# Autodesk Inventor assembly: Claw
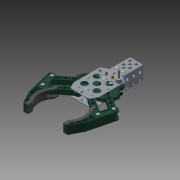
[picture p0: Inventor's stored thumbnail of the model, 180x180]
Saved by Autodesk Inventor 2016 SP2 (Build 200236200, 236)
## iProperties
Company: Microsoft
Created: 2014-02-04
Part Number: Claw
Description: STEP AP203
Document SubType Name: Assembly
Designer: Jacob
Sending System: SolidWorks 2013
Preprocessor: SwSTEP 2.0
Title: 276-2212.STEP
Author: svradm
Revision Number: ANY
## Documents named in this file (16)
- D:\Users\Owner\Desktop\Inventor Files\VEX Parts\Imperial\Motion\Claw.iam
- D:\Users\Owner\Desktop\Inventor Files\VEX Parts\Imperial\Motion\Components\VexLite-Claw-Brk RevA.ipt
- D:\Users\Owner\Desktop\Inventor Files\VEX Parts\Imperial\Motion\Components\BEARING-FLAT.ipt
- D:\Users\Owner\Desktop\Inventor Files\VEX Parts\Imperial\Motion\Components\CLAW-GEAR-LINKAGE.ipt
- D:\Users\Owner\Desktop\Inventor Files\VEX Parts\Imperial\Motion\Components\CLAW-LINKAGE.ipt
- D:\Users\Owner\Desktop\Inventor Files\VEX Parts\Imperial\Motion\Components\CLAW-LINKAGE-1.ipt
- D:\Users\Owner\Desktop\Inventor Files\VEX Parts\Imperial\Motion\Components\halfinch-Standoff.ipt
- D:\Users\Owner\Desktop\Inventor Files\VEX Parts\Imperial\Motion\Components\CLAW-FINGER.iam
- D:\Users\Owner\Desktop\Inventor Files\VEX Parts\Imperial\Motion\Components\rivet-outside.ipt
- D:\Users\Owner\Desktop\Inventor Files\VEX Parts\Imperial\Motion\Components\rivet-inside.ipt
- D:\Users\Owner\Desktop\Inventor Files\VEX Parts\Imperial\Motion\Components\VEX-12-TOOTH-GEAR.ipt
- D:\Users\Owner\Desktop\Inventor Files\VEX Parts\Imperial\Motion\Components\SHAFT-2000.ipt
- D:\Users\Owner\Desktop\Inventor Files\VEX Parts\Imperial\Motion\Components\SHAFT-COLLAR.ipt
- D:\Users\Owner\Desktop\Inventor Files\VEX Parts\Imperial\Motion\Components\SCREW-832-0250.ipt
- D:\Users\Owner\Desktop\Inventor Files\VEX Parts\Imperial\Motion\Components\SCREW-632-0250.ipt
- D:\Users\Owner\Desktop\Inventor Files\VEX Parts\Imperial\Motion\Components\ClawPinsLONG.iam
## Components (38 placed, 31 different names)
1. VexLite-Claw-Brk RevA_1 — Insert:5, Mate:4, Insert:6, Insert:9, Insert:10, Insert:13, Mate:12
2. VexLite-Claw-Brk RevA_2 — Mate:2, Mate:8, Mate:9, Mate:10, Mate:14
3. BEARING-FLAT_3
4. CLAW-GEAR-LINKAGE_4 — Mate:1, Insert:1, Mate:2, Mate:3, Rotation:1
5. CLAW-GEAR-LINKAGE_5 — Mate:6, Insert:7, Mate:8, Mate:9, Rotation:1, Rotation:2
6. CLAW-LINKAGE_6 — Mate:7, Insert:8, Mate:10, Mate:11
7. CLAW-LINKAGE-1_7 — Insert:2, Mate:4, Mate:5
8. halfinch-Standoff_8
9. halfinch-Standoff_9
10. halfinch-Standoff_10
11. halfinch-Standoff_11
12. CLAW-FINGER_28 [sub-assembly] — Mate:1, Insert:1, Insert:2, Insert:3, Insert:4
13. CLAW-FINGER_29 [sub-assembly] — Mate:6, Insert:7, Mate:7, Insert:8, Insert:11, Insert:12
14. rivet-outside_30
15. rivet-outside_31
16. rivet-inside_32
17. rivet-inside_33
18. VEX-12-TOOTH-GEAR_34 — Mate:14, Angle:1, Mate:15, Mate:16, Rotation:2
19. SCREW-832-0250_37
20. SCREW-832-0250_38
21. SCREW-832-0250_39
22. SCREW-832-0250_40
23. SCREW-832-0250_41
24. SCREW-832-0250_42
25. SCREW-832-0250_43
26. SCREW-832-0250_44
27. SCREW-632-0250_46
28. SCREW-632-0250_47
29. ClawPinsLONG:1 [sub-assembly] — Insert:3
30. ClawPinsLONG:2 [sub-assembly] — Insert:4
31. ClawPinsLONG:3 [sub-assembly] — Insert:5, Mate:3
32. ClawPinsLONG:4 [sub-assembly] — Insert:6, Mate:5
33. ClawPinsLONG:5 [sub-assembly] — Insert:9, Mate:11
34. ClawPinsLONG:6 [sub-assembly] — Insert:10
35. ClawPinsLONG:7 [sub-assembly] — Insert:11
36. ClawPinsLONG:8 [sub-assembly] — Insert:12
37. SHAFT-COLLAR:2 — Mate:12, Mate:13
38. SHAFT-2000:2 — Insert:13, Mate:13, Angle:1, Mate:15, Mate:16
## Relationships (32: Mate 16, Insert 13, RelateRotation 2, Angle 1)
- Mate:1: CLAW-GEAR-LINKAGE_4 ↔ CLAW-FINGER_28
- Insert:1: CLAW-GEAR-LINKAGE_4 ↔ CLAW-FINGER_28
- Insert:2: CLAW-LINKAGE-1_7 ↔ CLAW-FINGER_28
- Insert:3: CLAW-FINGER_28 ↔ ClawPinsLONG:1
- Insert:4: CLAW-FINGER_28 ↔ ClawPinsLONG:2
- Mate:2: VexLite-Claw-Brk RevA_2 ↔ CLAW-GEAR-LINKAGE_4
- Insert:5: VexLite-Claw-Brk RevA_1 ↔ ClawPinsLONG:3
- Mate:3: CLAW-GEAR-LINKAGE_4 ↔ ClawPinsLONG:3
- Mate:4: VexLite-Claw-Brk RevA_1 ↔ CLAW-LINKAGE-1_7
- Insert:6: VexLite-Claw-Brk RevA_1 ↔ ClawPinsLONG:4
- Mate:5: CLAW-LINKAGE-1_7 ↔ ClawPinsLONG:4
- Mate:6: CLAW-GEAR-LINKAGE_5 ↔ CLAW-FINGER_29
- Insert:7: CLAW-GEAR-LINKAGE_5 ↔ CLAW-FINGER_29
- Mate:7: CLAW-LINKAGE_6 ↔ CLAW-FINGER_29
- Insert:8: CLAW-LINKAGE_6 ↔ CLAW-FINGER_29
- Insert:9: VexLite-Claw-Brk RevA_1 ↔ ClawPinsLONG:5
- Insert:10: VexLite-Claw-Brk RevA_1 ↔ ClawPinsLONG:6
- Mate:8: VexLite-Claw-Brk RevA_2 ↔ CLAW-GEAR-LINKAGE_5
- Mate:9: VexLite-Claw-Brk RevA_2 ↔ CLAW-GEAR-LINKAGE_5
- Mate:10: VexLite-Claw-Brk RevA_2 ↔ CLAW-LINKAGE_6
- Mate:11: CLAW-LINKAGE_6 ↔ ClawPinsLONG:5
- Insert:11: CLAW-FINGER_29 ↔ ClawPinsLONG:7
- Insert:12: CLAW-FINGER_29 ↔ ClawPinsLONG:8
- Insert:13 (-21.0312 mm): VexLite-Claw-Brk RevA_1 ↔ SHAFT-2000:2
- Mate:12: VexLite-Claw-Brk RevA_1 ↔ SHAFT-COLLAR:2
- Mate:13: SHAFT-COLLAR:2 ↔ SHAFT-2000:2
- Mate:14: VexLite-Claw-Brk RevA_2 ↔ VEX-12-TOOTH-GEAR_34
- Angle:1 (0 deg): VEX-12-TOOTH-GEAR_34 ↔ SHAFT-2000:2
- Mate:15: VEX-12-TOOTH-GEAR_34 ↔ SHAFT-2000:2
- Mate:16: VEX-12-TOOTH-GEAR_34 ↔ SHAFT-2000:2
- Rotation:1 [RelateRotation] (1 ul): CLAW-GEAR-LINKAGE_4 ↔ CLAW-GEAR-LINKAGE_5
- Rotation:2 [RelateRotation] (0.3333 ul): CLAW-GEAR-LINKAGE_5 ↔ VEX-12-TOOTH-GEAR_34
